# Autodesk Inventor assembly: 조립품1
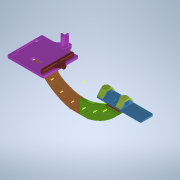
[picture p0: Inventor's stored thumbnail of the model, 180x180]
Saved by Autodesk Inventor 2021 (Build 250183000, 183)
## iProperties
Created: 2021-04-17
Part Number: 조립품1
Document SubType Name: Assembly
Designer: Dongyoon
Author: Dongyoon
## Documents named in this file (8)
- C:\Users\Dongyoon\Desktop\외주\첫번째-태양광\모델링\조립품1.iam
- C:\Users\Dongyoon\Desktop\외주\첫번째-태양광\모델링\Sun1.ipt
- C:\Users\Dongyoon\Desktop\외주\첫번째-태양광\모델링\sun2.ipt
- C:\Users\Dongyoon\Desktop\외주\첫번째-태양광\모델링\sun3.ipt
- C:\Users\Dongyoon\Desktop\외주\첫번째-태양광\모델링\sun4-1.ipt
- C:\Users\Dongyoon\Desktop\외주\첫번째-태양광\모델링\sun4-2.ipt
- C:\Users\Dongyoon\Desktop\외주\첫번째-태양광\모델링\wiper.ipt
- C:\Users\Dongyoon\Desktop\외주\첫번째-태양광\모델링\sun4-3.ipt
## Components (8 placed, 7 different names)
1. Sun1:1 — 메이트:7
2. sun2:1 — 메이트:1, 메이트:2, 플러쉬:1, 메이트:3, 플러쉬:2, 메이트:4, 플러쉬:5, 메이트:8, 메이트:12
3. sun3:1 — 메이트:1, 메이트:2, 플러쉬:1
4. sun3:2 — 메이트:3, 플러쉬:2, 메이트:4
5. sun4-1:1 — 메이트:5, 플러쉬:3, 플러쉬:4, 메이트:7
6. sun4-2:1 — 메이트:5, 플러쉬:3, 플러쉬:4, 플러쉬:5, 메이트:9, 메이트:10, 메이트:11
7. wiper:1 — 메이트:8
8. sun4-3:1 — 메이트:9, 메이트:10, 메이트:11, 메이트:12
## Relationships (16: Mate 11, Flush 5)
- 메이트:1 [Mate]: sun2:1 ↔ sun3:1
- 메이트:2 [Mate]: sun2:1 ↔ sun3:1
- 플러쉬:1 [Flush]: sun2:1 ↔ sun3:1
- 메이트:3 [Mate]: sun2:1 ↔ sun3:2
- 플러쉬:2 [Flush]: sun2:1 ↔ sun3:2
- 메이트:4 [Mate]: sun2:1 ↔ sun3:2
- 메이트:5 [Mate]: sun4-1:1 ↔ sun4-2:1
- 플러쉬:3 [Flush]: sun4-1:1 ↔ sun4-2:1
- 플러쉬:4 [Flush]: sun4-1:1 ↔ sun4-2:1
- 메이트:7 [Mate]: Sun1:1 ↔ sun4-1:1
- 플러쉬:5 [Flush]: sun2:1 ↔ sun4-2:1
- 메이트:8 [Mate] (155 mm): sun2:1 ↔ wiper:1
- 메이트:9 [Mate]: sun4-2:1 ↔ sun4-3:1
- 메이트:10 [Mate]: sun4-2:1 ↔ sun4-3:1
- 메이트:11 [Mate]: sun4-2:1 ↔ sun4-3:1
- 메이트:12 [Mate]: sun2:1 ↔ sun4-3:1
